# Autodesk Inventor assembly: 20 part layout
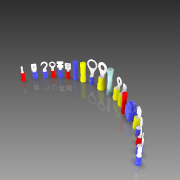
[picture p0: Inventor's stored thumbnail of the model, 180x180]
Saved by Autodesk Inventor 2014 (Build 180170000, 170)
## iProperties
Created: 2013-07-21
Part Number: 20 part layout
Document SubType Name: Assembly
Designer: Saville
Mass: 6.31285 g
Surface Area: 197.172 cm^2
Volume: 6.31285 cm^3
Density: 1 g/cm^3
Author: Saville
## Documents named in this file (21)
- C:\electrical nuts\terminal\20 part layout.iam
- C:\electrical nuts\cad\TERMINAL\17-64 yellow.ipt
- C:\electrical nuts\cad\TERMINAL\18-14 inline splice blue.ipt
- C:\electrical nuts\cad\TERMINAL\22-16 female flat spade red.ipt
- C:\electrical nuts\cad\TERMINAL\22-16 flat spade red.ipt
- C:\electrical nuts\cad\TERMINAL\22-18 double sided femal tube blue.ipt
- C:\electrical nuts\cad\TERMINAL\point 39 round blue.ipt
- C:\electrical nuts\cad\TERMINAL\point 091 male pin red.ipt
- C:\electrical nuts\cad\TERMINAL\point 107 double sided femal tube blue.ipt
- C:\electrical nuts\cad\TERMINAL\point 195 red round.ipt
- C:\electrical nuts\cad\TERMINAL\point 248 flat spade male.ipt
- C:\electrical nuts\cad\TERMINAL\12-10 circle yellow.ipt
- C:\electrical nuts\cad\TERMINAL\12-10 double sided female tube yellow.ipt
- C:\electrical nuts\cad\TERMINAL\12-10 female flat spade yellow.ipt
- C:\electrical nuts\cad\TERMINAL\13-64 hook blue.ipt
- C:\electrical nuts\cad\TERMINAL\13-64 u shape blue.ipt
- C:\electrical nuts\cad\TERMINAL\16-14 circle blue.ipt
- C:\electrical nuts\cad\TERMINAL\16-14 double sided femal tube heat shrink.ipt
- C:\electrical nuts\cad\TERMINAL\16-14 female spade blue.ipt
- C:\electrical nuts\cad\TERMINAL\16-14 male pin blue.ipt
- C:\electrical nuts\cad\TERMINAL\16-14 male spade blue.ipt
## Components (20 placed, 20 different names)
1. 17-64 yellow:1 — Mate:17
2. 18-14 inline splice blue:1 — Mate:16
3. 22-16 female flat spade red:1 — Mate:15
4. 22-16 flat spade red:1 — Mate:14
5. 22-18 double sided femal tube blue:1 — Mate:13
6. point 39 round blue:1 — Mate:12
7. point 091 male pin red:1 — Mate:11
8. point 107 double sided femal tube blue:1 — Mate:10
9. point 195 red round:1 — Mate:9
10. point 248 flat spade male:1 — Mate:8
11. 12-10 circle yellow:1 — Mate:7
12. 12-10 double sided female tube yellow:1 — Mate:6
13. 12-10 female flat spade yellow:1 — Mate:5
14. 13-64 hook blue:1 — Mate:18
15. 13-64 u shape blue:1 — Mate:19
16. 16-14 circle blue:1 — Mate:20
17. 16-14 double sided femal tube heat shrink:1 — Mate:4
18. 16-14 female spade blue:1 — Mate:3
19. 16-14 male pin blue:1 — Mate:2
20. 16-14 male spade blue:1 — Mate:1
## Relationships (20: Mate 20)
- Mate:1: 16-14 male spade blue:1
- Mate:2: 16-14 male pin blue:1
- Mate:3: 16-14 female spade blue:1
- Mate:4: 16-14 double sided femal tube heat shrink:1
- Mate:5: 12-10 female flat spade yellow:1
- Mate:6: 12-10 double sided female tube yellow:1
- Mate:7: 12-10 circle yellow:1
- Mate:8: point 248 flat spade male:1
- Mate:9: point 195 red round:1
- Mate:10: point 107 double sided femal tube blue:1
- Mate:11: point 091 male pin red:1
- Mate:12: point 39 round blue:1
- Mate:13: 22-18 double sided femal tube blue:1
- Mate:14: 22-16 flat spade red:1
- Mate:15: 22-16 female flat spade red:1
- Mate:16: 18-14 inline splice blue:1
- Mate:17: 17-64 yellow:1
- Mate:18: 13-64 hook blue:1
- Mate:19: 13-64 u shape blue:1
- Mate:20: 16-14 circle blue:1
